# Autodesk Inventor assembly: Urnenanlage 70 Ohne Denkmal
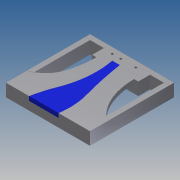
[picture p0: Inventor's stored thumbnail of the model, 180x180]
Saved by Autodesk Inventor 2014 (Build 180170000, 170)
## iProperties
Created: 2014-07-02
Part Number: Urnenanlage 70 Ohne Denkmal
Document SubType Name: Assembly
Designer: Semenov
Author: Semenov
## Documents named in this file (6)
- W:\DATEN_INVENTOR\LiTHOS_FORMEN\UA-070\Urnenanlage 70 Ohne Denkmal.iam
- W:\DATEN_INVENTOR\LiTHOS_FORMEN\UA-070\UA-70 EinfassungKT.ipt
- W:\DATEN_INVENTOR\LiTHOS_FORMEN\UA-070\UA-70 Sockel.ipt
- W:\DATEN_INVENTOR\LiTHOS_FORMEN\UA-070\UA-70 EinfassungST.ipt
- W:\DATEN_INVENTOR\LiTHOS_FORMEN\UA-070\UA-70 Platten aussen.ipt
- W:\DATEN_INVENTOR\LiTHOS_FORMEN\UA-070\UA-70 Platten mitte.ipt
## Components (5 placed, 5 different names)
1. UA-70 EinfassungKT:1 — Passend:1, Fluchtend:1, Fluchtend:2, Passend:2, Fluchtend:3, Fluchtend:4, Passend:3, Fluchtend:5, Fluchtend:6, Passend:4, Fluchtend:7, Fluchtend:8
2. UA-70 Sockel:1 — Passend:1, Fluchtend:1, Fluchtend:2
3. UA-70 EinfassungST:1 — Passend:2, Fluchtend:3, Fluchtend:4
4. UA-70 Platten aussen:1 — Passend:3, Fluchtend:5, Fluchtend:6
5. UA-70 Platten mitte:1 — Passend:4, Fluchtend:7, Fluchtend:8
## Relationships (12: Flush 8, Mate 4)
- Passend:1 [Mate]: UA-70 EinfassungKT:1 ↔ UA-70 Sockel:1
- Fluchtend:1 [Flush]: UA-70 EinfassungKT:1 ↔ UA-70 Sockel:1
- Fluchtend:2 [Flush]: UA-70 EinfassungKT:1 ↔ UA-70 Sockel:1
- Passend:2 [Mate]: UA-70 EinfassungKT:1 ↔ UA-70 EinfassungST:1
- Fluchtend:3 [Flush]: UA-70 EinfassungKT:1 ↔ UA-70 EinfassungST:1
- Fluchtend:4 [Flush]: UA-70 EinfassungKT:1 ↔ UA-70 EinfassungST:1
- Passend:3 [Mate]: UA-70 EinfassungKT:1 ↔ UA-70 Platten aussen:1
- Fluchtend:5 [Flush]: UA-70 EinfassungKT:1 ↔ UA-70 Platten aussen:1
- Fluchtend:6 [Flush]: UA-70 EinfassungKT:1 ↔ UA-70 Platten aussen:1
- Passend:4 [Mate]: UA-70 EinfassungKT:1 ↔ UA-70 Platten mitte:1
- Fluchtend:7 [Flush]: UA-70 EinfassungKT:1 ↔ UA-70 Platten mitte:1
- Fluchtend:8 [Flush]: UA-70 EinfassungKT:1 ↔ UA-70 Platten mitte:1
